# Autodesk Inventor assembly: Delb_Tail_Male(fr)
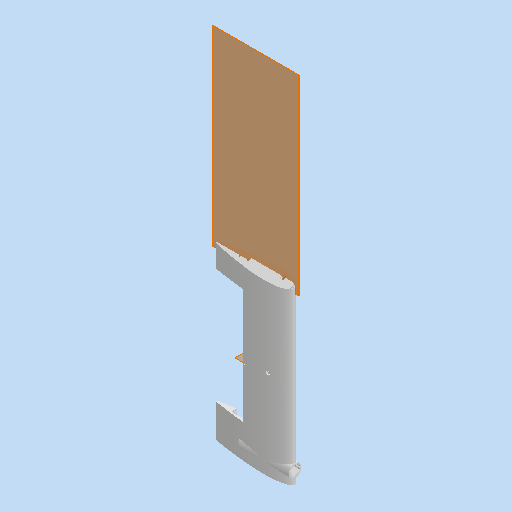
[picture p0: Inventor's stored thumbnail of the model, 512x512]
Saved by Autodesk Inventor 2027 (Build 310192060, 192F)
## iProperties
Created: 2026-08-06
Part Number: Delb_Tail_Male(fr)
Document SubType Name: Assembly
Designer: Delbe
Author: Delbe
## Documents named in this file (4)
- C:\GitHub\SWIFT-UAV\System_development\Pelican\structural_model\v0.3.0\Parts\Delb_Parts\Old_Models_and_Mich\Delb_Tail_Male(fr).iam
- C:\GitHub\SWIFT-UAV\System_development\Pelican\structural_model\v0.3.0\Parts\Delb_Parts\connector.ipt
- C:\GitHub\SWIFT-UAV\System_development\Pelican\structural_model\v0.3.0\Parts\Delb_Parts\Male_Tail_Female_Connector.ipt
- C:\GitHub\SWIFT-UAV\System_development\Pelican\structural_model\v0.3.0\Parts\Delb_Parts\Male_Tail_Male_Connector.ipt
## Components (3 placed, 3 different names)
1. connector:1 — Rigid:1
2. Male_Tail_Female_Connector:1 — Rigid:1, Rigid:2
3. Male_Tail_Male_Connector:1 — Rigid:2
## Relationships (2: WeldJoint 2)
- Rigid:1 [WeldJoint]: connector:1 ↔ Male_Tail_Female_Connector:1
- Rigid:2 [WeldJoint]: Male_Tail_Female_Connector:1 ↔ Male_Tail_Male_Connector:1
